# Autodesk Inventor assembly: Carcasa_Soldada
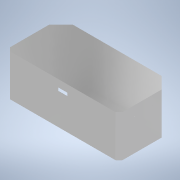
[picture p0: Inventor's stored thumbnail of the model, 180x180]
Saved by Autodesk Inventor 2022.1 (Build 261234000, 234)
## iProperties
Created: 2021-10-29
Part Number: Carcasa_Soldada
Document SubType Name: Weldment
Designer: seb_0
Weld Material: Welded Aluminum-6061
Author: seb_0
## Documents named in this file (2)
- C:\Users\seb_0\Desktop\PDM\ProyectoRobotPallet\Carcasa\Carcasa_v2.iam
- C:\Users\seb_0\Desktop\PDM\ProyectoRobotPallet\Carcasa\Carcasa.ipt
## Components (1 placed, 1 different names)
1. Carcasa:1 — Coincidencia:1, Coincidencia:2
## Relationships (2: Mate 2)
- Coincidencia:1 [Mate]: Carcasa:1
- Coincidencia:2 [Mate]: Carcasa:1
